# Autodesk Inventor assembly: ENSAMBLE_BALSA_UNDIMOTRIZ
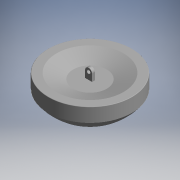
[picture p0: Inventor's stored thumbnail of the model, 180x180]
Saved by Autodesk Inventor 2019.4 (Build 234330000, 330)
## iProperties
Part Number: ENSAMBLE_BALSA_UNDIMOTRIZ
Document SubType Name: Ensamblaje
Designer: crist
Author: crist
## Documents named in this file (4)
- C:\Users\crist\Desktop\BALSA_UNDIMOTRIZ\ENSAMBLE_BALSA_UNDIMOTRIZ.iam
- C:\Users\crist\Desktop\BALSA_UNDIMOTRIZ\PARTE_INFERIOR_BALSA_FLOTABILIDAD_UNDIMOTRIZ.ipt
- C:\Users\crist\Desktop\BALSA_UNDIMOTRIZ\PARTE_SUPERIOR_BALSA_FLOTABILIDAD_UNIDMOTRIZVALPO.ipt
- C:\Users\crist\Desktop\BALSA_UNDIMOTRIZ\SUJECION_BALSA_UNDIMOTRIZ.ipt
## Components (3 placed, 3 different names)
1. PARTE_INFERIOR_BALSA_FLOTABILIDAD_UNDIMOTRIZ:1 — De rotación:1
2. PARTE_SUPERIOR_BALSA_FLOTABILIDAD_UNIDMOTRIZVALPO:1 — De rotación:1, Rígido:1
3. SUJECION_BALSA_UNDIMOTRIZ:1 — Rígido:1
## Relationships (2: RevoluteJoint 1, WeldJoint 1)
- De rotación:1 [RevoluteJoint]: PARTE_INFERIOR_BALSA_FLOTABILIDAD_UNDIMOTRIZ:1 ↔ PARTE_SUPERIOR_BALSA_FLOTABILIDAD_UNIDMOTRIZVALPO:1
- Rígido:1 [WeldJoint]: PARTE_SUPERIOR_BALSA_FLOTABILIDAD_UNIDMOTRIZVALPO:1 ↔ SUJECION_BALSA_UNDIMOTRIZ:1
